# Autodesk Inventor assembly: Poste de travail
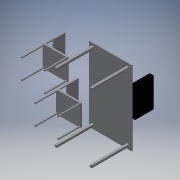
[picture p0: Inventor's stored thumbnail of the model, 180x180]
Saved by Autodesk Inventor 2016 SP1 (Build 200210100, 210)
## iProperties
Created: 2016-10-04
Part Number: Poste de travail
Material: Générique
Document SubType Name: Assembly
Designer: dimercur
EcartPiedChaise: 100,000 mm
ChaiseAvancée: 300,000 mm
ChaiseReculée: 550,000 mm
Author: dimercur
## Documents named in this file (4)
- D:\Users\dimercur\Documents\SVN\projets-gei\Salle 22-24\Poste de travail.iam
- D:\Users\dimercur\Documents\SVN\projets-gei\Salle 22-24\Chaise.ipt
- D:\Users\dimercur\Documents\SVN\projets-gei\Salle 22-24\Table.ipt
- D:\Users\dimercur\Documents\SVN\projets-gei\Salle 22-24\Ecran.ipt
## Components (4 placed, 3 different names)
1. Chaise:1 — Affleurement:1, Placage:2, Placage:3
2. Chaise:2 — Affleurement:2, Placage:1, Placage:4
3. Table:1 — Affleurement:1, Affleurement:2, Placage:1, Placage:2, Placage:3, Placage:4, Placage:5, Placage:6
4. Ecran:1 — Placage:5, Placage:6
## Relationships (8: Mate 6, Flush 2)
- Affleurement:1 [Flush]: Chaise:1 ↔ Table:1
- Affleurement:2 [Flush]: Chaise:2 ↔ Table:1
- Placage:1 [Mate] (100 mm): Chaise:2 ↔ Table:1
- Placage:2 [Mate] (100 mm): Chaise:1 ↔ Table:1
- Placage:3 [Mate] (300 mm): Chaise:1 ↔ Table:1
- Placage:4 [Mate] (550 mm): Chaise:2 ↔ Table:1
- Placage:5 [Mate]: Table:1 ↔ Ecran:1
- Placage:6 [Mate] (50 mm): Table:1 ↔ Ecran:1
